# Autodesk Inventor assembly: enc-BackPanel Top V2 - Assembly
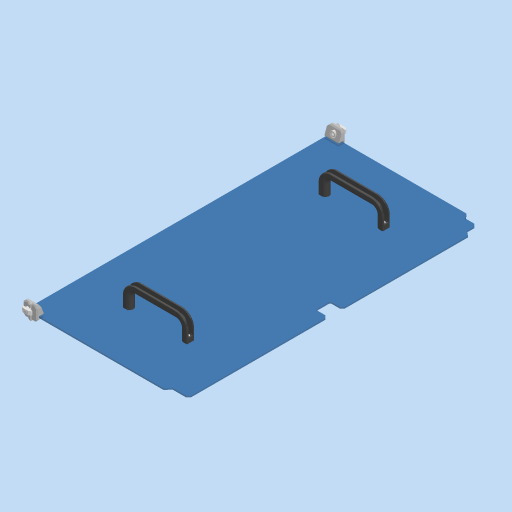
[picture p0: Inventor's stored thumbnail of the model, 512x512]
Saved by Autodesk Inventor 2023.2 (Build 272271000, 271)
## iProperties
Created: 2023-12-04
Part Number: enc-BackPanel Top V2 - Assembly
Document SubType Name: Assembly
Designer: Nils Bade
Author: Nils Bade
## Documents named in this file (4)
- C:\Users\nilsb\Documents\Inventor\Projektarbeit-Bade\Enclosure\enc-BackPanel Top V2 - Assembly.iam
- C:\Users\nilsb\Documents\Inventor\Projektarbeit-Bade\Enclosure\Panel Mount Vertical Guide for 4040 - Assembly.iam
- C:\Users\nilsb\Documents\Inventor\Projektarbeit-Bade\Enclosure\enc-BackPanel Top V2.ipt
- C:\Users\nilsb\Documents\Inventor\Projektarbeit-Bade\Enclosure\item_Handgriff_PA120_Assembly.iam
## Components (5 placed, 3 different names)
1. enc-BackPanel Top V2 for 4040 - 338x628:1 — Fluchtend:29, Passend:29, Passend:30, Passend:31, Passend:32, Passend:33, Passend:34
2. Panel Mount Vertical Guide for 4040 - Assembly:1 [sub-assembly] — Fluchtend:30
3. Panel Mount Vertical Guide for 4040 - Assembly:2 [sub-assembly] — Fluchtend:29, Fluchtend:30
4. item_Handgriff_120er:1 [sub-assembly] — Passend:29, Passend:30, Passend:34
5. item_Handgriff_120er:2 [sub-assembly] — Passend:31, Passend:32, Passend:33
## Relationships (12: Mate 10, Flush 2)
- [Mate]: enc-BackPanel Top V2 for 4040 - 338x628:1 ↔ Panel Mount Vertical Guide for 4040 - Assembly:2
- [Mate] (2 mm): enc-BackPanel Top V2 for 4040 - 338x628:1 ↔ Panel Mount Vertical Guide for 4040 - Assembly:2
- [Mate]: enc-BackPanel Top V2 for 4040 - 338x628:1 ↔ Panel Mount Vertical Guide for 4040 - Assembly:1
- [Mate] (2 mm): enc-BackPanel Top V2 for 4040 - 338x628:1 ↔ Panel Mount Vertical Guide for 4040 - Assembly:1
- Fluchtend:29 [Flush] (298 mm): enc-BackPanel Top V2 for 4040 - 338x628:1 ↔ Panel Mount Vertical Guide for 4040 - Assembly:2
- Passend:29 [Mate]: enc-BackPanel Top V2 for 4040 - 338x628:1 ↔ item_Handgriff_120er:1
- Passend:30 [Mate]: enc-BackPanel Top V2 for 4040 - 338x628:1 ↔ item_Handgriff_120er:1
- Passend:31 [Mate]: enc-BackPanel Top V2 for 4040 - 338x628:1 ↔ item_Handgriff_120er:2
- Passend:32 [Mate]: enc-BackPanel Top V2 for 4040 - 338x628:1 ↔ item_Handgriff_120er:2
- Passend:33 [Mate]: enc-BackPanel Top V2 for 4040 - 338x628:1 ↔ item_Handgriff_120er:2
- Passend:34 [Mate]: enc-BackPanel Top V2 for 4040 - 338x628:1 ↔ item_Handgriff_120er:1
- Fluchtend:30 [Flush]: Panel Mount Vertical Guide for 4040 - Assembly:1 ↔ Panel Mount Vertical Guide for 4040 - Assembly:2
